# Autodesk Inventor assembly: Rod Holder D
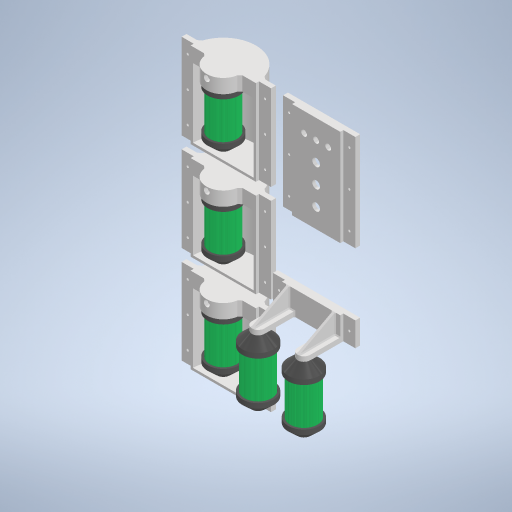
[picture p0: Inventor's stored thumbnail of the model, 512x512]
Saved by Autodesk Inventor 2024 (Build 280153020, 153B)
## iProperties
Created: 2023-08-02
Part Number: Rod Holder D
Document SubType Name: Assembly
Designer: torban
Author: torban
## Documents named in this file (5)
- D:\GIT\CIRC-2023-Night-Task-HW-SW\CAD\Reactor Control Panel\Rod Holder D.iam
- D:\GIT\CIRC-2023-Night-Task-HW-SW\CAD\Reactor\Reactor\Full.iam
- D:\GIT\CIRC-2023-Night-Task-HW-SW\CAD\Reactor Control Panel\Faceplate.ipt
- D:\GIT\CIRC-2023-Night-Task-HW-SW\CAD\Reactor Module\Reactor Module\Reactor Rod Holder Positions.iam
- D:\GIT\CIRC-2023-Night-Task-HW-SW\CAD\Reactor Control Panel\Rod Holder.iam
## Components (6 placed, 4 different names)
1. Full:1 [sub-assembly] — Mate:1, Flush:2, Flush:3
2. Full:2 [sub-assembly] — Mate:2, Flush:1, Flush:4, Flush:5, Flush:10
3. Full:3 [sub-assembly] — Mate:1, Mate:2, Flush:1, Flush:2, Flush:3, Flush:4, Mate:3, Flush:9
4. Faceplate:1 — Flush:5, Mate:3, Flush:7, Flush:8, Flush:10
5. Reactor Rod Holder Positions:1 [sub-assembly] — Mate:4, Mate:5, Mate:6
6. Rod Holder:1 [sub-assembly] — Flush:7, Flush:8, Mate:4, Mate:5, Mate:6, Flush:9
## Relationships (15: Flush 9, Mate 6)
- Mate:1 (25 mm): Full:1 ↔ Full:3
- Mate:2 (25 mm): Full:2 ↔ Full:3
- Flush:1: Full:2 ↔ Full:3
- Flush:2: Full:1 ↔ Full:3
- Flush:3: Full:1 ↔ Full:3
- Flush:4: Full:2 ↔ Full:3
- Flush:5: Full:2 ↔ Faceplate:1
- Mate:3 (25 mm): Full:3 ↔ Faceplate:1
- Flush:7: Faceplate:1 ↔ Rod Holder:1
- Flush:8: Faceplate:1 ↔ Rod Holder:1
- Mate:4: Reactor Rod Holder Positions:1 ↔ Rod Holder:1
- Mate:5: Reactor Rod Holder Positions:1 ↔ Rod Holder:1
- Mate:6: Reactor Rod Holder Positions:1 ↔ Rod Holder:1
- Flush:9: Full:3 ↔ Rod Holder:1
- Flush:10: Full:2 ↔ Faceplate:1
